# Autodesk Inventor assembly: Baterij.ipt
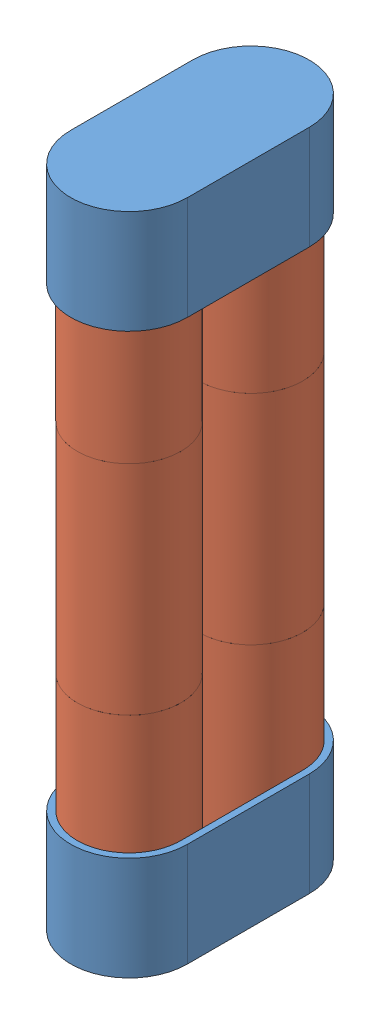
[picture p0: shaded view drawn from the part files that the assembly names]
Saved by Autodesk Inventor 2015 (Build 190159000, 159)
## iProperties
Created: 2016-01-04
Part Number: Baterij.ipt
Document SubType Name: Assembly
Designer: david
Author: david
## Documents named in this file (3)
- Z:\gip\Inventor\generatie 7\Frame\Electronica\Baterij\Baterij.ipt.iam
- Z:\gip\Inventor\generatie 7\Frame\Electronica\Baterij\Dopje.ipt
- Z:\gip\Inventor\generatie 7\Frame\Electronica\Baterij\Cell.ipt
## Components (8 placed, 2 different names)
1. Dopje:1 — Mate:1, Mate:2, Mate:3, Mate:4
2. Cell:1 — Mate:1, Mate:4, Mate:5, Mate:7
3. Cell:2 — Mate:2, Mate:3, Mate:6, Mate:8
4. Cell:3 — Mate:5, Mate:7, Mate:10, Mate:11
5. Cell:4 — Mate:6, Mate:8, Mate:9, Mate:12
6. Cell:5 — Mate:10, Mate:11, Mate:13, Mate:15
7. Cell:6 — Mate:9, Mate:12, Mate:14
8. Dopje:2 — Mate:13, Mate:14, Mate:15
## Relationships (15: Mate 15)
- Mate:1: Dopje:1 ↔ Cell:1
- Mate:2: Dopje:1 ↔ Cell:2
- Mate:3: Dopje:1 ↔ Cell:2
- Mate:4: Dopje:1 ↔ Cell:1
- Mate:5: Cell:1 ↔ Cell:3
- Mate:6: Cell:2 ↔ Cell:4
- Mate:7: Cell:1 ↔ Cell:3
- Mate:8: Cell:2 ↔ Cell:4
- Mate:9: Cell:4 ↔ Cell:6
- Mate:10: Cell:3 ↔ Cell:5
- Mate:11: Cell:3 ↔ Cell:5
- Mate:12: Cell:4 ↔ Cell:6
- Mate:13: Cell:5 ↔ Dopje:2
- Mate:14: Cell:6 ↔ Dopje:2
- Mate:15: Cell:5 ↔ Dopje:2
